# Autodesk Inventor assembly: __Case
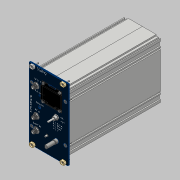
[picture p0: Inventor's stored thumbnail of the model, 180x180]
Saved by Autodesk Inventor 2021.4 (Build 254397000, 397)
## iProperties
Created: 2021-12-10
Part Number: __Case
Document SubType Name: Assembly
Designer: Tilman Preuschoff
Author: Tilman Preuschoff
## Documents named in this file (13)
- C:\Users\Tilman Preuschoff\Documents\GitHub\RF_frequency_modulator\frontpanel\assembly\__Case.iam
- C:\Users\Tilman Preuschoff\Documents\GitHub\RF_frequency_modulator\frontpanel\Fischer_TFP.ipt
- C:\Users\Tilman Preuschoff\Documents\GitHub\RF_frequency_modulator\frontpanel\assembly\display.ipt
- C:\Users\Tilman Preuschoff\Documents\GitHub\RF_frequency_modulator\frontpanel\assembly\MTS_module\RF_frequency_modulator.iam
- C:\Users\Tilman Preuschoff\Documents\GitHub\RF_frequency_modulator\frontpanel\assembly\9533ncdk_-_9100-9200-9500.iam
- C:\Users\Tilman Preuschoff\Documents\GitHub\RF_frequency_modulator\frontpanel\assembly\Potentiometer_Bourns_3005_Horizontal.ipt
- C:\Users\Tilman Preuschoff\Documents\GitHub\RF_frequency_modulator\frontpanel\assembly\KY-040 Rotary Encoder.ipt
- C:\Users\Tilman Preuschoff\Documents\GitHub\RF_frequency_modulator\frontpanel\assembly\5230_-_5000_-_panel.iam
- C:\Users\Tilman Preuschoff\Documents\GitHub\RF_frequency_modulator\frontpanel\assembly\Fischer HB.ipt
- C:\Users\Tilman Preuschoff\Documents\Inventor\Content Center Files\R2021\de-DE\BS EN ISO 7046-2 H\BS EN ISO 7046-2 H - M3x10 - 8.8 - H1.ipt
- C:\Users\Tilman Preuschoff\Documents\Inventor\Content Center Files\R2021\de-DE\DIN 84\DIN 84 - M2,5 x 6.ipt
- C:\Users\Tilman Preuschoff\Documents\Inventor\Content Center Files\R2021\de-DE\DIN 7985 (H)\DIN 7985 (H) - M2,5x10-H.ipt
- C:\Users\Tilman Preuschoff\Documents\GitHub\RF_frequency_modulator\frontpanel\assembly\KN1.ipt
## Components (25 placed, 12 different names)
1. Fischer HB:3 — Passend:1, Passend:2, Passend:3, Passend:6, Winkel:1, Drehbar:1, Passend:7, Fluchtend:2, Passend:11, Passend:12, Winkel:3
2. Fischer_TFP:1 — Passend:6, Winkel:1, Drehbar:1, Passend:8, Winkel:2, Passend:10, Passend:13, Drehbar:2, Drehbar:3, Starr:2, Drehbar:5, Drehbar:6, Drehbar:7, Drehbar:8, Drehbar:9, Drehbar:15, Drehbar:16, Drehbar:17, Drehbar:18
3. Fischer HB:4 — Passend:7, Passend:8, Fluchtend:2
4. display:1 — Winkel:2, Passend:13, Drehbar:2, Drehbar:10, Drehbar:12, Drehbar:13, Drehbar:14
5. RF_frequency_modulator:1 [sub-assembly] — Passend:10, Passend:11, Passend:12, Passend:17, Starr:1
6. 9533ncdk_-_9100-9200-9500:1 [sub-assembly] — Drehbar:3
7. Potentiometer_Bourns_3005_Horizontal:1 — Passend:17, Winkel:3, Starr:1
8. KY-040 Rotary Encoder:1 — Starr:2
9. 5230_-_5000_-_panel:1 [sub-assembly] — Drehbar:5
10. BS EN ISO 7046-2 H M3x10 - 8.8 - H1:1 — Drehbar:6
11. BS EN ISO 7046-2 H M3x10 - 8.8 - H1:2 — Drehbar:7
12. BS EN ISO 7046-2 H M3x10 - 8.8 - H1:3 — Drehbar:8
13. BS EN ISO 7046-2 H M3x10 - 8.8 - H1:4 — Drehbar:9
14. DIN 84 - ersetzt durch DIN EN ISO 1207 M2,5 x 6:1 — Drehbar:12
15. DIN 84 - ersetzt durch DIN EN ISO 1207 M2,5 x 6:2 — Drehbar:10
16. DIN 84 - ersetzt durch DIN EN ISO 1207 M2,5 x 6:3 — Drehbar:14
17. DIN 84 - ersetzt durch DIN EN ISO 1207 M2,5 x 6:4 — Drehbar:13
18. DIN 7985 (H) M2,5x10-H:1 — Drehbar:20
19. DIN 7985 (H) M2,5x10-H:2 — Drehbar:19
20. DIN 7985 (H) M2,5x10-H:3 — Drehbar:22
21. DIN 7985 (H) M2,5x10-H:4 — Drehbar:21
22. KN1:1 — Drehbar:15, Drehbar:19
23. KN1:2 — Drehbar:17, Drehbar:21
24. KN1:3 — Drehbar:16, Drehbar:20
25. KN1:4 — Drehbar:18, Drehbar:22
## Relationships (37: RevoluteJoint 20, Mate 11, Angle 3, WeldJoint 2, Flush 1)
- Passend:1 [Mate]: Fischer HB:3
- Passend:2 [Mate]: Fischer HB:3
- Passend:3 [Mate]: Fischer HB:3
- Passend:6 [Mate]: Fischer HB:3 ↔ Fischer_TFP:1
- Winkel:1 [Angle] (180 deg): Fischer HB:3 ↔ Fischer_TFP:1
- Drehbar:1 [RevoluteJoint]: Fischer HB:3 ↔ Fischer_TFP:1
- Passend:7 [Mate]: Fischer HB:3 ↔ Fischer HB:4
- Passend:8 [Mate]: Fischer_TFP:1 ↔ Fischer HB:4
- Fluchtend:2 [Flush]: Fischer HB:3 ↔ Fischer HB:4
- Winkel:2 [Angle] (0 deg): Fischer_TFP:1 ↔ display:1
- Passend:10 [Mate]: Fischer_TFP:1 ↔ RF_frequency_modulator:1
- Passend:11 [Mate]: Fischer HB:3 ↔ RF_frequency_modulator:1
- Passend:12 [Mate]: Fischer HB:3 ↔ RF_frequency_modulator:1
- Passend:13 [Mate]: Fischer_TFP:1 ↔ display:1
- Drehbar:2 [RevoluteJoint]: Fischer_TFP:1 ↔ display:1
- Drehbar:3 [RevoluteJoint]: Fischer_TFP:1 ↔ 9533ncdk_-_9100-9200-9500:1
- Passend:17 [Mate]: RF_frequency_modulator:1 ↔ Potentiometer_Bourns_3005_Horizontal:1
- Winkel:3 [Angle] (0 deg): Fischer HB:3 ↔ Potentiometer_Bourns_3005_Horizontal:1
- Starr:1 [WeldJoint]: RF_frequency_modulator:1 ↔ Potentiometer_Bourns_3005_Horizontal:1
- Starr:2 [WeldJoint]: Fischer_TFP:1 ↔ KY-040 Rotary Encoder:1
- Drehbar:5 [RevoluteJoint]: Fischer_TFP:1 ↔ 5230_-_5000_-_panel:1
- Drehbar:6 [RevoluteJoint]: Fischer_TFP:1 ↔ BS EN ISO 7046-2 H M3x10 - 8.8 - H1:1
- Drehbar:7 [RevoluteJoint]: Fischer_TFP:1 ↔ BS EN ISO 7046-2 H M3x10 - 8.8 - H1:2
- Drehbar:8 [RevoluteJoint]: Fischer_TFP:1 ↔ BS EN ISO 7046-2 H M3x10 - 8.8 - H1:3
- Drehbar:9 [RevoluteJoint]: Fischer_TFP:1 ↔ BS EN ISO 7046-2 H M3x10 - 8.8 - H1:4
- Drehbar:10 [RevoluteJoint]: display:1 ↔ DIN 84 - ersetzt durch DIN EN ISO 1207 M2,5 x 6:2
- Drehbar:12 [RevoluteJoint]: display:1 ↔ DIN 84 - ersetzt durch DIN EN ISO 1207 M2,5 x 6:1
- Drehbar:13 [RevoluteJoint]: display:1 ↔ DIN 84 - ersetzt durch DIN EN ISO 1207 M2,5 x 6:4
- Drehbar:14 [RevoluteJoint]: display:1 ↔ DIN 84 - ersetzt durch DIN EN ISO 1207 M2,5 x 6:3
- Drehbar:15 [RevoluteJoint]: Fischer_TFP:1 ↔ KN1:1
- Drehbar:16 [RevoluteJoint]: Fischer_TFP:1 ↔ KN1:3
- Drehbar:17 [RevoluteJoint]: Fischer_TFP:1 ↔ KN1:2
- Drehbar:18 [RevoluteJoint]: Fischer_TFP:1 ↔ KN1:4
- Drehbar:19 [RevoluteJoint]: DIN 7985 (H) M2,5x10-H:2 ↔ KN1:1
- Drehbar:20 [RevoluteJoint]: DIN 7985 (H) M2,5x10-H:1 ↔ KN1:3
- Drehbar:21 [RevoluteJoint]: DIN 7985 (H) M2,5x10-H:4 ↔ KN1:2
- Drehbar:22 [RevoluteJoint]: DIN 7985 (H) M2,5x10-H:3 ↔ KN1:4
